# Autodesk Inventor assembly: electric_asm
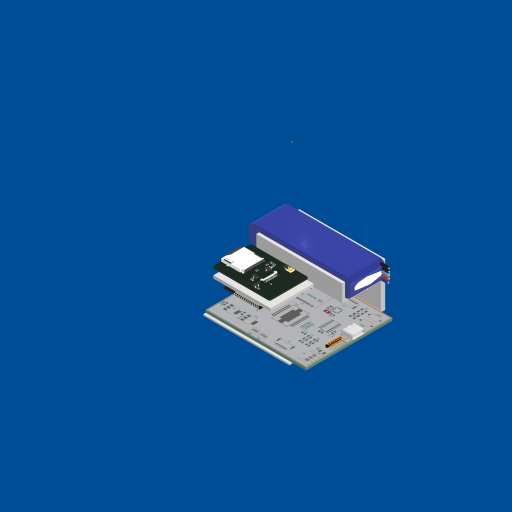
[picture p0: Inventor's stored thumbnail of the model, 512x512]
Saved by Autodesk Inventor 2023.1 (Build 271208000, 208)
## iProperties
Created: 2023-06-05
Part Number: electric_asm
Document SubType Name: Assembly
Designer: nara atthama
Author: nara atthama
## Documents named in this file (5)
- C:\Users\naraa\OneDrive - Universitas Airlangga\Dokumen\kuliah\MATKUL\sem6\TopSus\masbrobot\model\electric_asm.iam
- C:\Users\naraa\OneDrive - Universitas Airlangga\Dokumen\kuliah\MATKUL\sem6\TopSus\masbrobot\model\electric_base.ipt
- C:\Users\naraa\OneDrive - Universitas Airlangga\Dokumen\kuliah\MATKUL\sem6\TopSus\masbrobot\model\turnigy-nanotech-950mah-2s-25-50c-lipo-1.snapshot.4\Battery.ipt
- C:\Users\naraa\OneDrive - Universitas Airlangga\Dokumen\kuliah\MATKUL\sem6\TopSus\masbrobot\model\masbrobot2.iam
- C:\Users\naraa\OneDrive - Universitas Airlangga\Dokumen\kuliah\MATKUL\sem6\TopSus\masbrobot\model\ai-thinker-esp32-cam-1.snapshot.1\ESP32-CAM-AI_Thinker.iam
## Components (4 placed, 4 different names)
1. electric_base:1 — Mate:1, Flush:1, Mate:2, Mate:3, Mate:4, Mate:5
2. Battery:1 — Mate:3, Mate:4
3. masbrobot2:1 [sub-assembly] — Mate:1, Flush:1, Mate:2
4. ESP32-CAM-AI_Thinker:1 [sub-assembly] — Mate:5
## Relationships (6: Mate 5, Flush 1)
- Mate:1: electric_base:1 ↔ masbrobot2:1
- Flush:1 (-10 mm): electric_base:1 ↔ masbrobot2:1
- Mate:2 (2 mm): electric_base:1 ↔ masbrobot2:1
- Mate:3: electric_base:1 ↔ Battery:1
- Mate:4: electric_base:1 ↔ Battery:1
- Mate:5: electric_base:1 ↔ ESP32-CAM-AI_Thinker:1
